# Autodesk Inventor assembly: persitaltic pump assembly
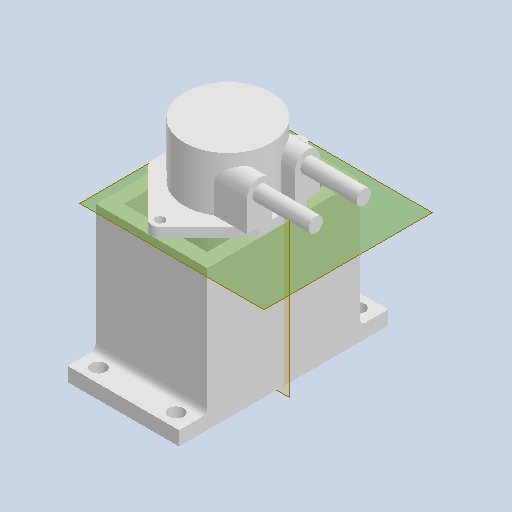
[picture p0: Inventor's stored thumbnail of the model, 512x512]
Saved by Autodesk Inventor 2022 (Build 260153000, 153)
## iProperties
Created: 2022-01-06
Part Number: persitaltic pump assembly
Document SubType Name: Assembly
Designer: efred
Author: efred
## Documents named in this file (3)
- C:\Users\efred\OneDrive - Imperial College London\ROBOICP\Final Assembly\persitaltic pump assembly.iam
- C:\Users\efred\OneDrive - Imperial College London\ROBOICP\Final Assembly\peristaltic pump.ipt
- C:\Users\efred\OneDrive - Imperial College London\ROBOICP\Final Assembly\peristaltic pump bracket.ipt
## Components (2 placed, 2 different names)
1. peristaltic pump:1 — Flush:1
2. peristaltic pump bracket:1 — Flush:2, Flush:3
## Relationships (3: Flush 3)
- Flush:1 (0.1 mm): peristaltic pump:1
- Flush:2: peristaltic pump bracket:1
- Flush:3: peristaltic pump bracket:1
